# Autodesk Inventor assembly: Assembly
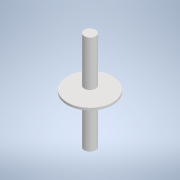
[picture p0: Inventor's stored thumbnail of the model, 180x180]
Saved by Autodesk Inventor 2022 (Build 260153000, 153)
## iProperties
Created: 2022-03-15
Part Number: Assembly
Document SubType Name: Assembly
Designer: kaebi
Author: kaebi
## Documents named in this file (3)
- C:\Users\kaebi\OneDrive - mci4me.at\03_MCI Master\4.Semester_SS2022\Masterarbeit\Software\CAD\Assembly.iam
- C:\Users\kaebi\OneDrive - mci4me.at\03_MCI Master\4.Semester_SS2022\Masterarbeit\Software\CAD\Bauteil_1.ipt
- C:\Users\kaebi\OneDrive - mci4me.at\03_MCI Master\4.Semester_SS2022\Masterarbeit\Software\CAD\Bauteil_2.ipt
## Components (3 placed, 2 different names)
1. Bauteil_1:1 — Passend:3, Passend:4, Passend:5
2. Bauteil_2:1 — Passend:1, Passend:2, Passend:3, Passend:4, Passend:6
3. Bauteil_1:2 — Passend:5, Passend:6
## Relationships (6: Mate 6)
- Passend:1 [Mate]: Bauteil_2:1
- Passend:2 [Mate]: Bauteil_2:1
- Passend:3 [Mate]: Bauteil_1:1 ↔ Bauteil_2:1
- Passend:4 [Mate] (1.5 mm): Bauteil_1:1 ↔ Bauteil_2:1
- Passend:5 [Mate]: Bauteil_1:1 ↔ Bauteil_1:2
- Passend:6 [Mate] (1 mm): Bauteil_2:1 ↔ Bauteil_1:2
## Named parameters: upperDistance = 1.5 mm, lowerDistance = 1 mm
